# Autodesk Inventor assembly: manipulator
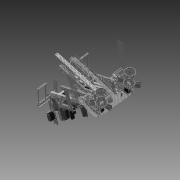
[picture p0: Inventor's stored thumbnail of the model, 180x180]
Saved by Autodesk Inventor 2014 SP1 (Build 180222100, 222)
## iProperties
Created: 2014-04-06
Part Number: manipulator
Document SubType Name: Assembly
Designer: Ryan
Author: Ryan
## Documents named in this file (8)
- C:\Users\Ryan\Desktop\sw\toss up 5th A bot\manipulator\manipulator.iam
- C:\Users\Ryan\Desktop\sw\toss up 5th A bot\6bar\6 bar_MIR.iam
- C:\Users\Ryan\Desktop\sw\toss up 5th A bot\6bar\6 bar.iam
- C:\Users\Ryan\Desktop\sw\toss up 5th A bot\intake\intake.iam
- C:\Users\Ryan\Desktop\sw\toss up 5th A bot\tower\tower.iam
- C:\Users\Ryan\Desktop\sw\toss up 5th A bot\tower\tower_MIR.iam
- C:\Users\Ryan\Desktop\sw\toss up 5th A bot\tower\buttons.iam
- C:\Users\Ryan\Desktop\sw\lib\Super Sonic Sparks VEX CAD Library\Other Parts\7.2V (Robot Battery) NiMH 3000mAh.ipt
## Components (8 placed, 7 different names)
1. 6 bar_MIR:1 [sub-assembly] — Mate:4, Mate:5, Mate:6, Mate:11, Mate:12, Mate:13
2. 6 bar:1 [sub-assembly] — Mate:1, Mate:2, Mate:3, Mate:7, Mate:9, Mate:14
3. intake:1 [sub-assembly] — Mate:1, Mate:2, Mate:3, Mate:4, Mate:5, Mate:6
4. tower:1 [sub-assembly] — Mate:7, Mate:9, Flush:1, Mate:14, Mate:16, Mate:17, Mate:19
5. tower_MIR:1 [sub-assembly] — Mate:11, Flush:1, Mate:12, Mate:13, Mate:15, Mate:18
6. buttons:1 [sub-assembly] — Mate:15, Mate:16, Mate:17, Mate:18, Angle:1
7. 7.2V (Robot Battery) NiMH 3000mAh:1 — Mate:19, Angle:1
8. 7.2V (Robot Battery) NiMH 3000mAh:2
## Component patterns: (2 elements, first: 7.2V (Robot Battery) NiMH 3000mAh:1)
## Relationships (19: Mate 17, Flush 1, Angle 1)
- Mate:1: 6 bar:1 ↔ intake:1
- Mate:2: 6 bar:1 ↔ intake:1
- Mate:3: 6 bar:1 ↔ intake:1
- Mate:4: 6 bar_MIR:1 ↔ intake:1
- Mate:5: 6 bar_MIR:1 ↔ intake:1
- Mate:6: 6 bar_MIR:1 ↔ intake:1
- Mate:7: 6 bar:1 ↔ tower:1
- Mate:9: 6 bar:1 ↔ tower:1
- Mate:11: 6 bar_MIR:1 ↔ tower_MIR:1
- Flush:1: tower:1 ↔ tower_MIR:1
- Mate:12: 6 bar_MIR:1 ↔ tower_MIR:1
- Mate:13: 6 bar_MIR:1 ↔ tower_MIR:1
- Mate:14: 6 bar:1 ↔ tower:1
- Mate:15: tower_MIR:1 ↔ buttons:1
- Mate:16 (2.3114 mm): tower:1 ↔ buttons:1
- Mate:17 (2.3114 mm): tower:1 ↔ buttons:1
- Mate:18 (2.3114 mm): tower_MIR:1 ↔ buttons:1
- Mate:19: tower:1 ↔ 7.2V (Robot Battery) NiMH 3000mAh:1
- Angle:1 (0 deg): buttons:1 ↔ 7.2V (Robot Battery) NiMH 3000mAh:1
## Named parameters: q = 2.3114 mm
